# Autodesk Inventor assembly: robot
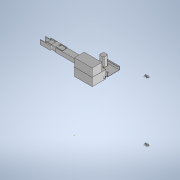
[picture p0: Inventor's stored thumbnail of the model, 180x180]
Saved by Autodesk Inventor 2020 (Build 240168000, 168)
## iProperties
Created: 2021-03-19
Part Number: robot
Document SubType Name: Assembly
Designer: super
Author: super
## Documents named in this file (5)
- C:\desk\promissionsave\inventor\robot\robot morango slider.iam
- C:\desk\promissionsave\inventor\robot\armj1.ipt
- C:\desk\promissionsave\inventor\robot\guia.ipt
- C:\desk\promissionsave\inventor\container\c150x43x15x600.ipt
- C:\desk\promissionsave\inventor\robot\robot morango-.iam
## Components (6 placed, 4 different names)
1. armj1:2 — Mate:13
2. armj1:3 — Mate:13
3. c150x43x15x600:1 — Mate:14
4. guia:3
5. guia:4
6. robot morango-:1 [sub-assembly] — Flush:1, Flush:2, Mate:14
## Relationships (4: Mate 2, Flush 2)
- Mate:13: armj1:2 ↔ armj1:3
- Flush:1: robot morango-:1
- Flush:2: robot morango-:1
- Mate:14: c150x43x15x600:1 ↔ robot morango-:1
